# Autodesk Inventor assembly: FullElevatorShart
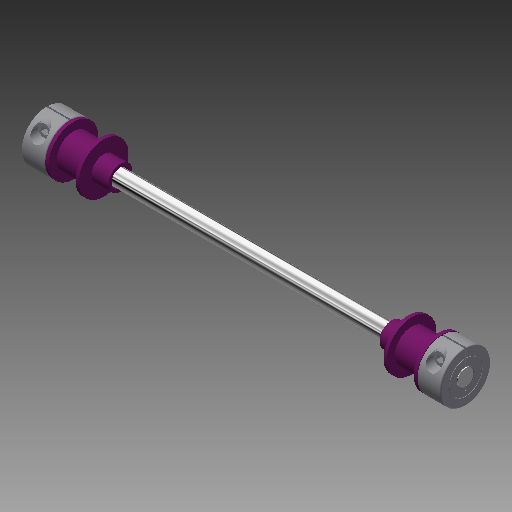
[picture p0: Inventor's stored thumbnail of the model, 512x512]
Saved by Autodesk Inventor 2019 (Build 230136000, 136)
## iProperties
Created: 2019-09-28
Part Number: FullElevatorShart
Document SubType Name: Assembly
Designer: james
Author: james
## Documents named in this file (4)
- F:\JimsDesign\Jims2020FTC\FullElevatorShart.iam
- F:\JimsDesign\Jims2020FTC\ElevatorShaft.ipt
- F:\JimsDesign\Library\McMaster\57445K230_ONE-PIECE CLAMP-ON SHAFT COLLAR.ipt
- F:\JimsDesign\Jims2020FTC\IdlePully.ipt
## Components (5 placed, 3 different names)
1. ElevatorShaft:1 — Mate:1, Mate:2, Flush:1, Flush:2, Mate:3, Mate:4
2. 57445K230_ONE-PIECE CLAMP-ON SHAFT COLLAR:1 — Mate:1, Flush:2, Mate:6
3. 57445K230_ONE-PIECE CLAMP-ON SHAFT COLLAR:2 — Mate:2, Flush:1, Mate:5
4. IdlePully:1 — Mate:4, Mate:5
5. IdlePully:2 — Mate:3, Mate:6
## Relationships (8: Mate 6, Flush 2)
- Mate:1: ElevatorShaft:1 ↔ 57445K230_ONE-PIECE CLAMP-ON SHAFT COLLAR:1
- Mate:2: ElevatorShaft:1 ↔ 57445K230_ONE-PIECE CLAMP-ON SHAFT COLLAR:2
- Flush:1: ElevatorShaft:1 ↔ 57445K230_ONE-PIECE CLAMP-ON SHAFT COLLAR:2
- Flush:2: ElevatorShaft:1 ↔ 57445K230_ONE-PIECE CLAMP-ON SHAFT COLLAR:1
- Mate:3: ElevatorShaft:1 ↔ IdlePully:2
- Mate:4: ElevatorShaft:1 ↔ IdlePully:1
- Mate:5: 57445K230_ONE-PIECE CLAMP-ON SHAFT COLLAR:2 ↔ IdlePully:1
- Mate:6: 57445K230_ONE-PIECE CLAMP-ON SHAFT COLLAR:1 ↔ IdlePully:2
